# Autodesk Inventor assembly: insertAssembly
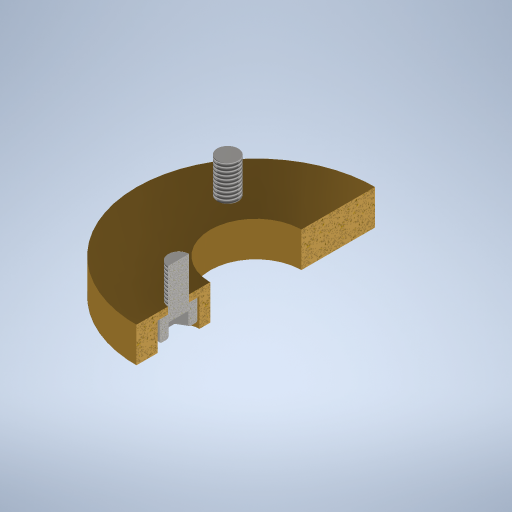
[picture p0: Inventor's stored thumbnail of the model, 512x512]
Saved by Autodesk Inventor 2024 (Build 280153000, 153)
## iProperties
Created: 2023-09-24
Part Number: insertAssembly
Document SubType Name: Assembly
Designer: schanen
Author: schanen
## Documents named in this file (3)
- C:\Users\schanen\Documents\Inventor\he4inserts\insertAssembly.iam
- C:\Users\schanen\Documents\Inventor\he4inserts\Insert_Top.ipt
- C:\Users\schanen\Documents\Inventor\he4inserts\Screw_StainlessSteal_M3_SocketCap_6mm.ipt
## Components (4 placed, 2 different names)
1. Insert_Top:1 — Mate:1, Mate:2, Mate:3, Mate:4, Mate:5
2. Screw_StainlessSteal_M3_SocketCap_6mm:3 — Mate:1, Mate:2
3. Screw_StainlessSteal_M3_SocketCap_6mm:4
4. Screw_StainlessSteal_M3_SocketCap_6mm:5
## Component patterns: (3 elements, first: Screw_StainlessSteal_M3_SocketCap_6mm:3)
## Relationships (5: Mate 5)
- Mate:1: Insert_Top:1 ↔ Screw_StainlessSteal_M3_SocketCap_6mm:3
- Mate:2: Insert_Top:1 ↔ Screw_StainlessSteal_M3_SocketCap_6mm:3
- Mate:3: Insert_Top:1
- Mate:4: Insert_Top:1
- Mate:5: Insert_Top:1
